# Autodesk Inventor assembly: MK4i Swerve Module L3
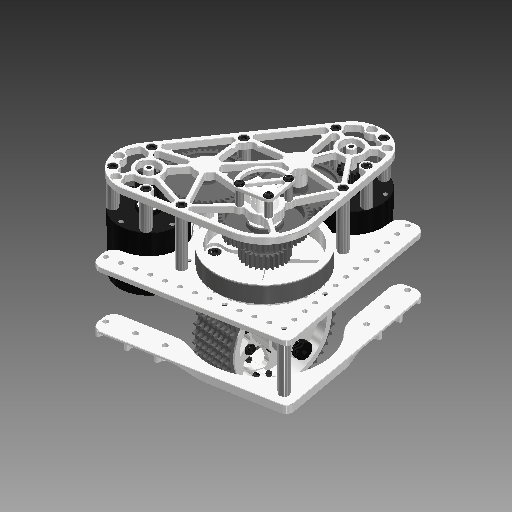
[picture p0: Inventor's stored thumbnail of the model, 512x512]
Saved by Autodesk Inventor 2025 (Build 290162010, 162A)
## iProperties
Created: 2024-07-19
Part Number: MK4i Swerve Module L3
Document SubType Name: Assembly
Designer: rohan
Author: rohan
## Documents named in this file (6)
- D:\ultimate-hecker\Computer-Aided-Design\FRC-Offseason-Design-Training\Parts Library\Drivetrains\Swerve Modules\MK4i\MK4i Swerve Module L3.iam
- D:\ultimate-hecker\Computer-Aided-Design\FRC-Offseason-Design-Training\Parts Library\Drivetrains\Swerve Modules\MK4i\MK4i Master Structure.iam
- D:\ultimate-hecker\Computer-Aided-Design\FRC-Offseason-Design-Training\Parts Library\Power Transfer\Belts and Pullies\320-5M-15 Belt.ipt
- D:\ultimate-hecker\Computer-Aided-Design\FRC-Offseason-Design-Training\Parts Library\Power Transfer\Gears (Hex)\50T 20DP Spur Gear 375 Hex (SDS).ipt
- D:\ultimate-hecker\Computer-Aided-Design\FRC-Offseason-Design-Training\Parts Library\Power Transfer\Gears (Motor)\SDS-Steel-Spur-Gear (20DP, 8mm Bore, 14T, 14T CD).ipt
- D:\ultimate-hecker\Computer-Aided-Design\FRC-Offseason-Design-Training\Parts Library\Drivetrains\Swerve Modules\MK4\MK4 Turret Assembly L3.iam
## Components (7 placed, 5 different names)
1. MK4i Master Structure:1 [sub-assembly] — Mate:1, Mate:2, Mate:3, Mate:4, Mate:5, Mate:6, Mate:7, Mate:8, Mate:9, Insert:2, Insert:3
2. MK4 Turret Assembly L3:1 [sub-assembly] — Mate:1, Mate:2, Insert:1, Rotation:3
3. 320-5M-15 Belt:1 — Insert:1, Mate:3
4. 50T 20DP Spur Gear 375 Hex (SDS):1 — Mate:4, Mate:5, Mate:6, Rotation:1, Rotation:3
5. 50T 20DP Spur Gear 375 Hex (SDS):2 — Mate:7, Mate:8, Mate:9, Rotation:2
6. SDS-Steel-Spur-Gear (20DP, 8mm Bore, 14T, 14T CD):1 — Insert:3, Rotation:1
7. SDS-Steel-Spur-Gear (20DP, 8mm Bore, 14T, 14T CD):2 — Insert:2, Rotation:2
## Relationships (15: Mate 9, Insert 3, RelateRotation 3)
- Mate:1: MK4i Master Structure:1 ↔ MK4 Turret Assembly L3:1
- Mate:2: MK4i Master Structure:1 ↔ MK4 Turret Assembly L3:1
- Insert:1 (1.016 mm): MK4 Turret Assembly L3:1 ↔ 320-5M-15 Belt:1
- Mate:3: MK4i Master Structure:1 ↔ 320-5M-15 Belt:1
- Mate:4: MK4i Master Structure:1 ↔ 50T 20DP Spur Gear 375 Hex (SDS):1
- Mate:5: MK4i Master Structure:1 ↔ 50T 20DP Spur Gear 375 Hex (SDS):1
- Mate:6: MK4i Master Structure:1 ↔ 50T 20DP Spur Gear 375 Hex (SDS):1
- Mate:7: MK4i Master Structure:1 ↔ 50T 20DP Spur Gear 375 Hex (SDS):2
- Mate:8: MK4i Master Structure:1 ↔ 50T 20DP Spur Gear 375 Hex (SDS):2
- Mate:9: MK4i Master Structure:1 ↔ 50T 20DP Spur Gear 375 Hex (SDS):2
- Insert:2: MK4i Master Structure:1 ↔ SDS-Steel-Spur-Gear (20DP, 8mm Bore, 14T, 14T CD):2
- Insert:3: MK4i Master Structure:1 ↔ SDS-Steel-Spur-Gear (20DP, 8mm Bore, 14T, 14T CD):1
- Rotation:1 [RelateRotation] (0.28 ul): 50T 20DP Spur Gear 375 Hex (SDS):1 ↔ SDS-Steel-Spur-Gear (20DP, 8mm Bore, 14T, 14T CD):1
- Rotation:2 [RelateRotation] (0.28 ul): 50T 20DP Spur Gear 375 Hex (SDS):2 ↔ SDS-Steel-Spur-Gear (20DP, 8mm Bore, 14T, 14T CD):2
- Rotation:3 [RelateRotation] (1 ul): MK4 Turret Assembly L3:1 ↔ 50T 20DP Spur Gear 375 Hex (SDS):1
